# Autodesk Inventor assembly: Assembly1
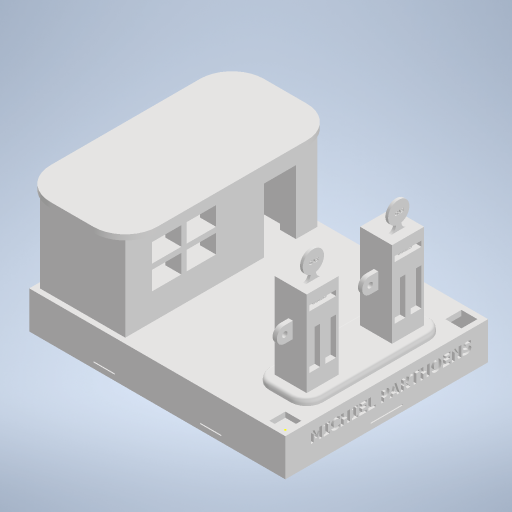
[picture p0: Inventor's stored thumbnail of the model, 512x512]
Saved by Autodesk Inventor 2023 (Build 270158000, 158)
## iProperties
Created: 2023-06-06
Part Number: Assembly1
Document SubType Name: Assembly
Designer: Prestige
Author: Prestige
## Documents named in this file (5)
- C:\Users\Prestige\Desktop\pxl\Semester 2 2022-2023\project ontwerpen\case design\design  1\Assembly1.iam
- C:\Users\Prestige\Desktop\pxl\Semester 2 2022-2023\project ontwerpen\case design\design  1\onderkant.ipt
- C:\Users\Prestige\Desktop\pxl\Semester 2 2022-2023\project ontwerpen\case design\design  1\bovenkant.ipt
- C:\Users\Prestige\Desktop\pxl\Semester 2 2022-2023\project ontwerpen\case design\design  1\gaspomp.ipt
- C:\Users\Prestige\Desktop\pxl\Semester 2 2022-2023\project ontwerpen\case design\design  1\huis.ipt
## Components (5 placed, 4 different names)
1. onderkant:1 — Flush:1, Flush:2, Flush:3
2. bovenkant:1 — Flush:1, Flush:2, Flush:3, Mate:1, Mate:2, Mate:3, Mate:4, Mate:5, Mate:6, Mate:7, Mate:8, Mate:9
3. gaspomp:1 — Mate:2, Mate:5, Mate:6
4. gaspomp:2 — Mate:1, Mate:3, Mate:4
5. huis:1 — Mate:7, Mate:8, Mate:9
## Relationships (12: Mate 9, Flush 3)
- Flush:1: onderkant:1 ↔ bovenkant:1
- Flush:2: onderkant:1 ↔ bovenkant:1
- Flush:3: onderkant:1 ↔ bovenkant:1
- Mate:1: bovenkant:1 ↔ gaspomp:2
- Mate:2: bovenkant:1 ↔ gaspomp:1
- Mate:3: bovenkant:1 ↔ gaspomp:2
- Mate:4: bovenkant:1 ↔ gaspomp:2
- Mate:5: bovenkant:1 ↔ gaspomp:1
- Mate:6: bovenkant:1 ↔ gaspomp:1
- Mate:7: bovenkant:1 ↔ huis:1
- Mate:8: bovenkant:1 ↔ huis:1
- Mate:9: bovenkant:1 ↔ huis:1
